# Autodesk Inventor assembly: Main_v6
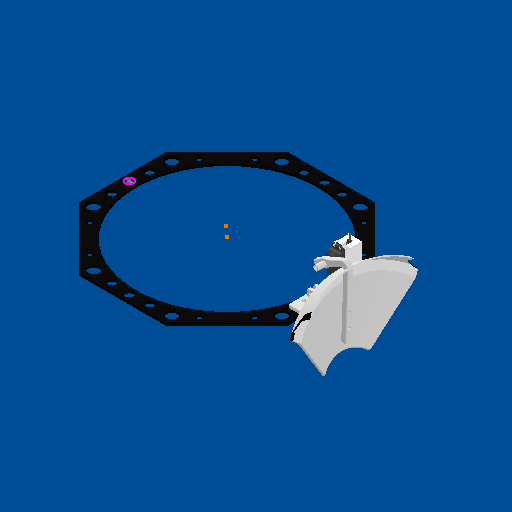
[picture p0: Inventor's stored thumbnail of the model, 512x512]
Saved by Autodesk Inventor 2026.2 (Build 302298000, 298)
## iProperties
Created: 2026-03-12
Part Number: Main_v6
Document SubType Name: Assembly
Designer: Thoma
Author: Thoma
## Documents named in this file (9)
- C:\Users\Thoma\OneDrive\Desktop\dir\telescope_cover\main\version_2\Main_v6.iam
- C:\Users\Thoma\OneDrive\Desktop\dir\telescope_cover\telescope\version_4\Telescope_End.ipt
- C:\Users\Thoma\OneDrive\Desktop\dir\telescope_cover\cover\base_plate_v18.ipt
- C:\Users\Thoma\OneDrive\Desktop\dir\telescope_cover\servo\DSS-M15S Servo.ipt
- C:\Users\Thoma\OneDrive\Desktop\dir\telescope_cover\cover\rod_v13.ipt
- C:\Users\Thoma\OneDrive\Desktop\dir\telescope_cover\cover\servo_attach_derive.ipt
- C:\Users\Thoma\OneDrive\Desktop\dir\telescope_cover\cover\Cover_Solo_v1.ipt
- C:\Users\Thoma\OneDrive\Desktop\dir\telescope_cover\cover\base_plate_bottom_v8.ipt
- C:\Users\Thoma\OneDrive\Desktop\dir\telescope_cover\servo\limit_switch_v2.ipt
## Components (8 placed, 8 different names)
1. Telescope_End:1 — Mate:1, Angle:1, Mate:2, Mate:13
2. base_plate_v18:1 — Mate:1, Angle:1, Mate:2, Mate:4, Mate:5, Mate:6, Mate:14, Mate:15, Mate:16, Mate:17, Flush:1
3. DSS-M15S Servo:1 — Mate:4, Mate:5, Mate:6, Mate:7, Mate:8
4. rod_v13:1 — Mate:9, Mate:10, Angle:2, Tangent:1, Mate:11, Mate:12
5. servo_attach_derive:1 — Mate:7, Mate:8, Mate:9, Mate:10, Angle:2
6. Cover_Solo_v1:1 — Tangent:1, Mate:11, Mate:12
7. base_plate_bottom_v8:1 — Mate:13, Mate:14, Mate:15
8. limit_switch_v2:1 — Mate:16, Mate:17, Flush:1
## Relationships (20: Mate 16, Angle 2, Tangent 1, Flush 1)
- Mate:1: Telescope_End:1 ↔ base_plate_v18:1
- Angle:1 (0 deg): Telescope_End:1 ↔ base_plate_v18:1
- Mate:2: Telescope_End:1 ↔ base_plate_v18:1
- Mate:4 (0.5 mm): base_plate_v18:1 ↔ DSS-M15S Servo:1
- Mate:5 (0.5 mm): base_plate_v18:1 ↔ DSS-M15S Servo:1
- Mate:6: base_plate_v18:1 ↔ DSS-M15S Servo:1
- Mate:7: DSS-M15S Servo:1 ↔ servo_attach_derive:1
- Mate:8: DSS-M15S Servo:1 ↔ servo_attach_derive:1
- Mate:9: rod_v13:1 ↔ servo_attach_derive:1
- Mate:10: rod_v13:1 ↔ servo_attach_derive:1
- Angle:2 (0 deg): rod_v13:1 ↔ servo_attach_derive:1
- Tangent:1 (-1 mm): rod_v13:1 ↔ Cover_Solo_v1:1
- Mate:11: rod_v13:1 ↔ Cover_Solo_v1:1
- Mate:12: rod_v13:1 ↔ Cover_Solo_v1:1
- Mate:13: Telescope_End:1 ↔ base_plate_bottom_v8:1
- Mate:14: base_plate_v18:1 ↔ base_plate_bottom_v8:1
- Mate:15: base_plate_v18:1 ↔ base_plate_bottom_v8:1
- Mate:16 (0.4 mm): base_plate_v18:1 ↔ limit_switch_v2:1
- Mate:17 (0.4 mm): base_plate_v18:1 ↔ limit_switch_v2:1
- Flush:1: base_plate_v18:1 ↔ limit_switch_v2:1
